# Autodesk Inventor assembly: pen plotter
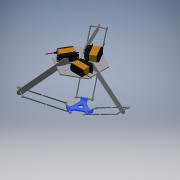
[picture p0: Inventor's stored thumbnail of the model, 180x180]
Saved by Autodesk Inventor 2016 (Build 200138000, 138)
## iProperties
Created: 2016-04-21
Part Number: pen plotter
Document SubType Name: Assembly
Designer: Sam
Author: Sam
## Documents named in this file (7)
- C:\Users\Sam\Documents\Arduino\Birobot\CAD\Inventor Files\pen plotter.iam
- C:\Users\Sam\Documents\Arduino\Birobot\CAD\Inventor Files\servo mount.ipt
- C:\Users\Sam\Documents\Arduino\Birobot\CAD\Inventor Files\FUTABA BLS251.iam
- C:\Users\Sam\Documents\Arduino\Birobot\CAD\Inventor Files\upper link.ipt
- C:\Users\Sam\Documents\Arduino\Birobot\CAD\Inventor Files\lower link assembly\crossbar.ipt
- C:\Users\Sam\Documents\Arduino\Birobot\CAD\Inventor Files\lower link assembly\longbar.ipt
- C:\Users\Sam\Documents\Arduino\Birobot\CAD\Inventor Files\end effector.ipt
## Components (20 placed, 6 different names)
1. servo mount:1 — Mate:1, Mate:2, Mate:3, Mate:4, Angle:1, Flush:1, Flush:2, Flush:3, Flush:4, Flush:5, Flush:6, Angle:8
2. FUTABA BLS251:1 [sub-assembly] — Mate:2, Angle:1, Flush:3, Flush:4, Insert:2
3. FUTABA BLS251:2 [sub-assembly] — Mate:3, Flush:1, Flush:5, Insert:3
4. FUTABA BLS251:3 [sub-assembly] — Mate:4, Flush:2, Flush:6, Mate:5, Insert:1
5. upper link:1 — Insert:2, Mate:6, Tangent:1
6. upper link:2 — Insert:3, Mate:7, Tangent:2
7. upper link:3 — Mate:5, Insert:1, Mate:8, Tangent:3
8. crossbar:1 — Mate:6, Tangent:1, Tangent:4, Tangent:5
9. crossbar:2 — Mate:7, Tangent:2, Tangent:8, Tangent:9
10. crossbar:3 — Mate:8, Tangent:3, Tangent:12, Tangent:13
11. longbar:1 — Tangent:4, Tangent:7, Angle:2
12. longbar:2 — Tangent:5, Tangent:6, Angle:2
13. longbar:3 — Tangent:9, Angle:3, Tangent:11
14. longbar:4 — Tangent:8, Angle:3, Tangent:10
15. longbar:5 — Tangent:12, Angle:4, Tangent:14
16. longbar:6 — Tangent:13, Angle:4, Tangent:15
17. crossbar:4 — Tangent:6, Tangent:7, Angle:6, Mate:10, Mate:12
18. crossbar:5 — Tangent:10, Tangent:11, Angle:5, Angle:7, Tangent:16, Flush:7
19. crossbar:6 — Tangent:14, Tangent:15, Angle:5, Mate:9, Mate:11
20. end effector:1 — Angle:6, Angle:7, Angle:8, Tangent:16, Mate:9, Mate:10, Flush:7, Mate:11, Mate:12
## Relationships (46: Tangent 16, Mate 12, Angle 8, Flush 7, Insert 3)
- Mate:1: servo mount:1
- Mate:2: servo mount:1 ↔ FUTABA BLS251:1
- Mate:3: servo mount:1 ↔ FUTABA BLS251:2
- Mate:4: servo mount:1 ↔ FUTABA BLS251:3
- Angle:1 (0 deg): servo mount:1 ↔ FUTABA BLS251:1
- Flush:1: servo mount:1 ↔ FUTABA BLS251:2
- Flush:2: servo mount:1 ↔ FUTABA BLS251:3
- Flush:3: servo mount:1 ↔ FUTABA BLS251:1
- Flush:4: servo mount:1 ↔ FUTABA BLS251:1
- Flush:5: servo mount:1 ↔ FUTABA BLS251:2
- Flush:6: servo mount:1 ↔ FUTABA BLS251:3
- Mate:5: FUTABA BLS251:3 ↔ upper link:3
- Insert:1: FUTABA BLS251:3 ↔ upper link:3
- Insert:2: FUTABA BLS251:1 ↔ upper link:1
- Insert:3: FUTABA BLS251:2 ↔ upper link:2
- Mate:6 (-0.65 mm): upper link:1 ↔ crossbar:1
- Tangent:1: upper link:1 ↔ crossbar:1
- Mate:7 (-0.65 mm): upper link:2 ↔ crossbar:2
- Tangent:2: upper link:2 ↔ crossbar:2
- Mate:8 (-0.65 mm): upper link:3 ↔ crossbar:3
- Tangent:3: upper link:3 ↔ crossbar:3
- Tangent:4: crossbar:1 ↔ longbar:1
- Tangent:5: crossbar:1 ↔ longbar:2
- Tangent:6: longbar:2 ↔ crossbar:4
- Tangent:7: longbar:1 ↔ crossbar:4
- Angle:2 (180 deg): longbar:1 ↔ longbar:2
- Tangent:8: crossbar:2 ↔ longbar:4
- Tangent:9: crossbar:2 ↔ longbar:3
- Angle:3 (180 deg): longbar:3 ↔ longbar:4
- Tangent:10: longbar:4 ↔ crossbar:5
- Tangent:11: longbar:3 ↔ crossbar:5
- Tangent:12: crossbar:3 ↔ longbar:5
- Tangent:13: crossbar:3 ↔ longbar:6
- Angle:4 (180 deg): longbar:5 ↔ longbar:6
- Tangent:14: longbar:5 ↔ crossbar:6
- Tangent:15: longbar:6 ↔ crossbar:6
- Angle:5 (60 deg): crossbar:5 ↔ crossbar:6
- Angle:6 (180 deg): crossbar:4 ↔ end effector:1
- Angle:7 (180 deg): crossbar:5 ↔ end effector:1
- Angle:8 (180 deg): servo mount:1 ↔ end effector:1
- Tangent:16: crossbar:5 ↔ end effector:1
- Mate:9: crossbar:6 ↔ end effector:1
- Mate:10: crossbar:4 ↔ end effector:1
- Flush:7 (-7.5 mm): crossbar:5 ↔ end effector:1
- Mate:11 (-7.5 mm): crossbar:6 ↔ end effector:1
- Mate:12 (-7.5 mm): crossbar:4 ↔ end effector:1
